# Autodesk Inventor assembly: Assy_cam_connection
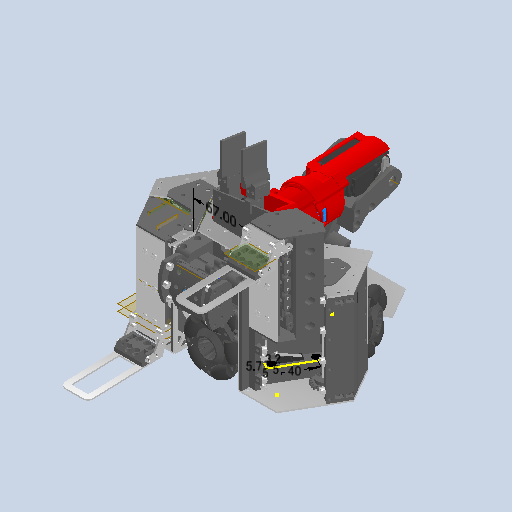
[picture p0: Inventor's stored thumbnail of the model, 512x512]
Saved by Autodesk Inventor 2024.1 (Build 281209000, 209)
## iProperties
Created: 2025-03-04
Part Number: Assy_cam_connection
Document SubType Name: Assembly
Designer: hibik
Author: hibik
## Documents named in this file (8)
- C:\Users\hibik\Documents\Robomech\RESCUE\ORCA\hard\Assy_cam_connection.iam
- C:\Users\hibik\Documents\Robomech\RESCUE\ORCA\hard\Assy_fork_connection.iam
- C:\Users\hibik\Documents\Robomech\RESCUE\ORCA\hard\arm\Assy_arm.iam
- C:\Users\hibik\Documents\Robomech\RESCUE\ORCA\hard\flame_front\cam_setter_left_under.ipt
- C:\Users\hibik\Documents\Robomech\RESCUE\ORCA\hard\flame_front\cam_setter_left_upper.ipt
- C:\Users\hibik\Documents\Robomech\RESCUE\ORCA\hard\flame_front\cam_setter_right_under.ipt
- C:\Users\hibik\Documents\Robomech\RESCUE\ORCA\hard\flame_front\cam_setter_right_upper.ipt
- C:\Users\hibik\Documents\Robomech\RESCUE\ORCA\hard\camera\cam_set.iam
## Components (7 placed, 7 different names)
1. Assy_fork_connection:1 [sub-assembly] — 挿入:8, 挿入:9, 挿入:11, 挿入:12, 角度:1
2. Assy_arm:1 [sub-assembly] — 挿入:8, 挿入:9
3. cam_setter_left_under:1 — 挿入:11, 挿入:14, 角度:2, 角度:3, 挿入:15
4. cam_setter_left_upper:1 — 挿入:16
5. cam_setter_right_under:1 — 挿入:12, 挿入:16
6. cam_setter_right_upper:1 — 挿入:15
7. cam_set:1 [sub-assembly] — 挿入:14, 角度:1, 角度:2, 角度:3
## Relationships (10: Insert 7, Angle 3)
- 挿入:8 [Insert]: Assy_fork_connection:1 ↔ Assy_arm:1
- 挿入:9 [Insert]: Assy_fork_connection:1 ↔ Assy_arm:1
- 挿入:11 [Insert]: Assy_fork_connection:1 ↔ cam_setter_left_under:1
- 挿入:12 [Insert]: Assy_fork_connection:1 ↔ cam_setter_right_under:1
- 挿入:14 [Insert]: cam_setter_left_under:1 ↔ cam_set:1
- 角度:1 [Angle] (0 deg): Assy_fork_connection:1 ↔ cam_set:1
- 角度:2 [Angle] (0 deg): cam_setter_left_under:1 ↔ cam_set:1
- 角度:3 [Angle] (0 deg): cam_setter_left_under:1 ↔ cam_set:1
- 挿入:15 [Insert]: cam_setter_left_under:1 ↔ cam_setter_right_upper:1
- 挿入:16 [Insert]: cam_setter_left_upper:1 ↔ cam_setter_right_under:1
